# Autodesk Inventor assembly: Body
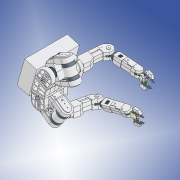
[picture p0: Inventor's stored thumbnail of the model, 180x180]
Saved by Autodesk Inventor 2017 (Build 210142000, 142)
## iProperties
Created: 2017-03-13
Part Number: Body
Document SubType Name: Assembly
Designer: zallen
Author: zallen
## Documents named in this file (4)
- C:\Users\zallen\Documents\GitHub\cr-laundry-robot\src\Body\Body.iam
- C:\Users\zallen\Documents\GitHub\cr-laundry-robot\src\Body\Arm Assembly\ArmAssembly.iam
- C:\Users\zallen\Documents\GitHub\cr-laundry-robot\src\Body\Chest Assembly\Chest Assembly.iam
- C:\Users\zallen\Documents\GitHub\cr-laundry-robot\src\Body\Spine Assembly\Spine Assembly.iam
## Components (4 placed, 3 different names)
1. ArmAssembly:1 [sub-assembly] — Mate:34, Mate:35, Mate:39
2. ArmAssembly:2 [sub-assembly] — Mate:19, Mate:32, Mate:40
3. Chest Assembly:1 [sub-assembly] — Mate:19, Mate:24, Mate:32, Mate:34, Mate:35, Mate:36, Mate:37, Mate:38, Mate:39, Mate:40
4. Spine Assembly:1 [sub-assembly] — Mate:24, Mate:36, Mate:37, Mate:38
## Relationships (10: Mate 10)
- Mate:19: ArmAssembly:2 ↔ Chest Assembly:1
- Mate:24: Chest Assembly:1 ↔ Spine Assembly:1
- Mate:32: ArmAssembly:2 ↔ Chest Assembly:1
- Mate:34: ArmAssembly:1 ↔ Chest Assembly:1
- Mate:35: ArmAssembly:1 ↔ Chest Assembly:1
- Mate:36: Chest Assembly:1 ↔ Spine Assembly:1
- Mate:37: Chest Assembly:1 ↔ Spine Assembly:1
- Mate:38: Chest Assembly:1 ↔ Spine Assembly:1
- Mate:39: ArmAssembly:1 ↔ Chest Assembly:1
- Mate:40: ArmAssembly:2 ↔ Chest Assembly:1
